# Autodesk Inventor assembly: Trianle box assembly
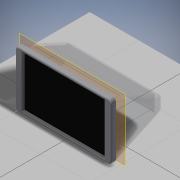
[picture p0: Inventor's stored thumbnail of the model, 180x180]
Saved by Autodesk Inventor 2018 (Build 220112000, 112)
## iProperties
Created: 2019-09-13
Part Number: Trianle box assembly
Document SubType Name: Assembly
Designer: Jacob
Author: Jacob
## Documents named in this file (7)
- C:\Users\Jacob\Documents\IPRO 497\Alarm box parts\Trianle box assembly.iam
- C:\Users\Jacob\Documents\IPRO 497\Alarm box parts\Triangle touch screen base.ipt
- C:\Users\Jacob\Documents\IPRO 497\Alarm box parts\Touch screen front box part.ipt
- C:\Users\Jacob\Documents\IPRO 497\Alarm box parts\raspberry pi display.ipt
- C:\Users\Jacob\Documents\IPRO 497\Alarm box parts\Official parts\raspberry pi display module.ipt
- C:\Users\Jacob\Documents\IPRO 497\Alarm box parts\Official parts\Stand off.ipt
- C:\Users\Jacob\Documents\IPRO 497\Alarm box parts\Official parts\Raspberry Pi 3 .ipt
## Components (9 placed, 6 different names)
1. Triangle touch screen base:1 — Mate:4, Mate:5, Mate:6
2. Touch screen front box part:1 — Mate:1, Mate:2, Mate:3, Mate:4, Mate:5, Mate:6
3. raspberry pi display:1 — Mate:1, Mate:2, Mate:3, Mate:7, Mate:8, Mate:9
4. raspberry pi display module:1 — Mate:7, Mate:8, Mate:9, Mate:10, Mate:11, Mate:12, Mate:13, Mate:14, Mate:15, Mate:16, Mate:17
5. Stand off:1 — Mate:10, Mate:11
6. Stand off:2 — Mate:16, Mate:17
7. Stand off:3 — Mate:14, Mate:15, Mate:20
8. Stand off:4 — Mate:12, Mate:13, Mate:18, Mate:19
9. Raspberry Pi 3 :1 — Mate:18, Mate:19, Mate:20
## Relationships (20: Mate 20)
- Mate:1: Touch screen front box part:1 ↔ raspberry pi display:1
- Mate:2: Touch screen front box part:1 ↔ raspberry pi display:1
- Mate:3: Touch screen front box part:1 ↔ raspberry pi display:1
- Mate:4: Triangle touch screen base:1 ↔ Touch screen front box part:1
- Mate:5: Triangle touch screen base:1 ↔ Touch screen front box part:1
- Mate:6: Triangle touch screen base:1 ↔ Touch screen front box part:1
- Mate:7: raspberry pi display:1 ↔ raspberry pi display module:1
- Mate:8: raspberry pi display:1 ↔ raspberry pi display module:1
- Mate:9: raspberry pi display:1 ↔ raspberry pi display module:1
- Mate:10: raspberry pi display module:1 ↔ Stand off:1
- Mate:11: raspberry pi display module:1 ↔ Stand off:1
- Mate:12: raspberry pi display module:1 ↔ Stand off:4
- Mate:13: raspberry pi display module:1 ↔ Stand off:4
- Mate:14: raspberry pi display module:1 ↔ Stand off:3
- Mate:15: raspberry pi display module:1 ↔ Stand off:3
- Mate:16: raspberry pi display module:1 ↔ Stand off:2
- Mate:17: raspberry pi display module:1 ↔ Stand off:2
- Mate:18: Stand off:4 ↔ Raspberry Pi 3 :1
- Mate:19: Stand off:4 ↔ Raspberry Pi 3 :1
- Mate:20: Stand off:3 ↔ Raspberry Pi 3 :1
